# Autodesk Inventor assembly: Manipulator
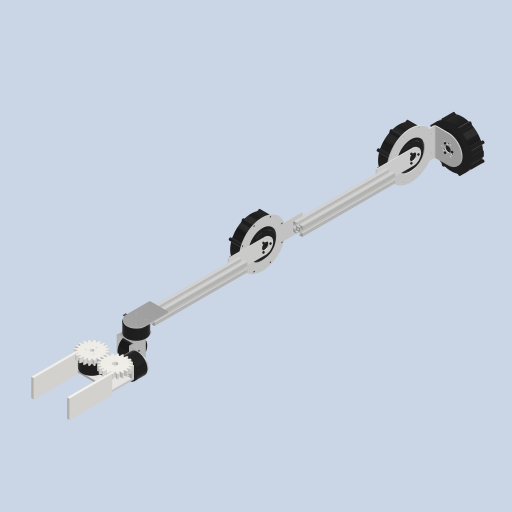
[picture p0: Inventor's stored thumbnail of the model, 512x512]
Saved by Autodesk Inventor 2023 (Build 270158000, 158)
## iProperties
Created: 2024-11-08
Part Number: Manipulator
Document SubType Name: Assembly
Designer: kiyo
Author: kiyo
## Documents named in this file (11)
- D:\GitHub\inventor\syu-si\OfficeRobot\Manipulator\Manipulator.iam
- D:\GitHub\inventor\syu-si\OfficeRobot\ReadyMade\Steadywin\GIM8108-8.iam
- D:\GitHub\inventor\syu-si\OfficeRobot\Manipulator\sholder-roll-bracket.ipt
- D:\GitHub\inventor\syu-si\OfficeRobot\Manipulator\shoulder_pitch_plate.ipt
- D:\GitHub\inventor\syu-si\OfficeRobot\Manipulator\elbow-pitch-bracket.ipt
- D:\GitHub\inventor\syu-si\OfficeRobot\Manipulator\HFS5-2020-200.ipt
- D:\GitHub\inventor\syu-si\OfficeRobot\Manipulator\Hand.iam
- D:\GitHub\inventor\syu-si\OfficeRobot\Manipulator\wrist-pitch-plate.ipt
- D:\GitHub\inventor\syu-si\OfficeRobot\Manipulator\wrist-yaw-plate.ipt
- D:\GitHub\inventor\syu-si\OfficeRobot\ReadyMade\Steadywin\GIM3505-8.ipt
- D:\GitHub\inventor\syu-si\OfficeRobot\Manipulator\wrist_roll_plate.ipt
## Components (16 placed, 10 different names)
1. GIM8108-8:1 [sub-assembly] — 挿入:1
2. GIM8108-8:2 [sub-assembly] — 挿入:2, 挿入:3, 挿入:4
3. GIM8108-8:3 [sub-assembly] — 挿入:5, 挿入:6, 挿入:7
4. sholder-roll-bracket:1 — 挿入:1, 挿入:2, 挿入:3, 肩ヨー
5. shoulder_pitch_plate:1 — 挿入:4, メイト:1, フラッシュ:1, メイト:2, 肩ピッチ
6. elbow-pitch-bracket:1 — メイト:3, メイト:4, フラッシュ:2, 挿入:5, 挿入:6
7. HFS5-2020-200:1 — メイト:1, フラッシュ:1, メイト:2, メイト:3, メイト:4, フラッシュ:2
8. shoulder_pitch_plate:2 — 挿入:7, 肘ピッチ
9. HFS5-2020-200:3 — メイト:7, メイト:8, フラッシュ:4
10. Hand:1 [sub-assembly] — 挿入:16, ハンド
11. wrist-pitch-plate:1 — 挿入:9, 挿入:11, 挿入:12, 手首ヨー
12. wrist-yaw-plate:1 — 挿入:8, メイト:7, メイト:8, フラッシュ:4, 挿入:10
13. GIM3505-8:1 — 挿入:8, 挿入:9, 挿入:10
14. GIM3505-8:2 — 挿入:11, 挿入:12, 挿入:13
15. GIM3505-8:3 — 挿入:14, 挿入:15, 挿入:16
16. wrist_roll_plate:1 — 挿入:13, 挿入:14, 挿入:15, 手首ピッチ
## Relationships (34: Insert 16, Mate 8, Angle 6, Flush 4)
- 挿入:1 [Insert]: GIM8108-8:1 ↔ sholder-roll-bracket:1
- 挿入:2 [Insert]: GIM8108-8:2 ↔ sholder-roll-bracket:1
- 挿入:3 [Insert]: GIM8108-8:2 ↔ sholder-roll-bracket:1
- 挿入:4 [Insert]: GIM8108-8:2 ↔ shoulder_pitch_plate:1
- メイト:1 [Mate]: shoulder_pitch_plate:1 ↔ HFS5-2020-200:1
- フラッシュ:1 [Flush] (6.5 mm): shoulder_pitch_plate:1 ↔ HFS5-2020-200:1
- メイト:2 [Mate] (-20 mm): shoulder_pitch_plate:1 ↔ HFS5-2020-200:1
- メイト:3 [Mate]: elbow-pitch-bracket:1 ↔ HFS5-2020-200:1
- メイト:4 [Mate] (-20 mm): elbow-pitch-bracket:1 ↔ HFS5-2020-200:1
- フラッシュ:2 [Flush] (-7 mm): elbow-pitch-bracket:1 ↔ HFS5-2020-200:1
- 挿入:5 [Insert]: GIM8108-8:3 ↔ elbow-pitch-bracket:1
- 挿入:6 [Insert]: GIM8108-8:3 ↔ elbow-pitch-bracket:1
- [Mate]: shoulder_pitch_plate:2 ↔ HFS5-2020-200:3
- [Flush] (6.5 mm): shoulder_pitch_plate:2 ↔ HFS5-2020-200:3
- [Mate] (-20 mm): shoulder_pitch_plate:2 ↔ HFS5-2020-200:3
- 挿入:7 [Insert]: GIM8108-8:3 ↔ shoulder_pitch_plate:2
- 挿入:8 [Insert]: wrist-yaw-plate:1 ↔ GIM3505-8:1
- メイト:7 [Mate]: HFS5-2020-200:3 ↔ wrist-yaw-plate:1
- メイト:8 [Mate] (-20 mm): HFS5-2020-200:3 ↔ wrist-yaw-plate:1
- フラッシュ:4 [Flush] (-10.5 mm): HFS5-2020-200:3 ↔ wrist-yaw-plate:1
- 挿入:9 [Insert]: wrist-pitch-plate:1 ↔ GIM3505-8:1
- 挿入:10 [Insert]: wrist-yaw-plate:1 ↔ GIM3505-8:1
- 挿入:11 [Insert]: wrist-pitch-plate:1 ↔ GIM3505-8:2
- 挿入:12 [Insert]: wrist-pitch-plate:1 ↔ GIM3505-8:2
- 挿入:13 [Insert]: GIM3505-8:2 ↔ wrist_roll_plate:1
- 挿入:14 [Insert]: GIM3505-8:3 ↔ wrist_roll_plate:1
- 挿入:15 [Insert]: GIM3505-8:3 ↔ wrist_roll_plate:1
- 挿入:16 [Insert]: Hand:1 ↔ GIM3505-8:3
- 肩ヨー [Angle] (0 deg): sholder-roll-bracket:1
- 肩ピッチ [Angle] (0 deg): shoulder_pitch_plate:1
- 肘ピッチ [Angle] (0 deg): shoulder_pitch_plate:2
- 手首ヨー [Angle] (0 deg): wrist-pitch-plate:1
- 手首ピッチ [Angle] (0 deg): wrist_roll_plate:1
- ハンド [Angle] (0 deg): Hand:1
## Named parameters: d12_d4 = 0 mm, d13_d5 = 6.5 mm, d14_d6 = -20 mm
